# Autodesk Inventor assembly: Sink cabinet
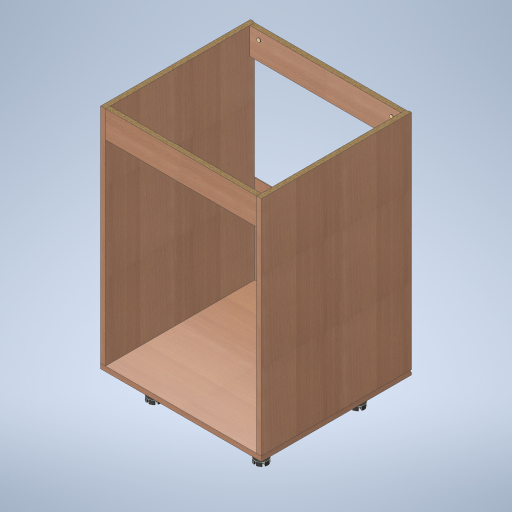
[picture p0: Inventor's stored thumbnail of the model, 512x512]
Saved by Autodesk Inventor 2024 (Build 280153000, 153)
## iProperties
RuleStatus: InUse
Created: 2017-01-27
Part Number: Sink cabinet
Document SubType Name: Assembly
Designer: SvetlanaB
Author: SvetlanaB
## Documents named in this file (17)
- C:\W4INV 2024 Design\iBOX LIBRARY\Kitchen\Standing Cabinets\Sink cabinet\Sink cabinet.iam
- C:\W4INV 2024 Design\iBOX LIBRARY\Kitchen\Standing Cabinets\Sink cabinet\Bottom panel.ipt
- C:\W4INV 2024 Design\iBOX LIBRARY\Kitchen\Standing Cabinets\Sink cabinet\Left panel.ipt
- C:\W4INV 2024 Design\iBOX LIBRARY\Kitchen\Standing Cabinets\Sink cabinet\Right panel.ipt
- C:\W4INV 2024 Design\iBOX LIBRARY\Kitchen\Standing Cabinets\Sink cabinet\Front panel.ipt
- C:\W4INV 2024 Design\iBOX LIBRARY\Kitchen\Standing Cabinets\Sink cabinet\Back top panel.ipt
- C:\W4INV 2024 Design\iBOX LIBRARY\Kitchen\Standing Cabinets\Sink cabinet\Back bottom panel.ipt
- C:\W4INV 2024 Design\_LIBRARY\Supports and legs\Legs\ADJUSTABLE LEG\Adjustable leg  BT18 clip included.ipt
- C:\W4INV 2024 Design\_LIBRARY\Supports and legs\Legs\ADJUSTABLE LEG\Adjustable leg  BT18.ipt
- C:\W4INV 2024 Design\_LIBRARY\Fixed joints\Confirmat\CONFIRMAT\Confirmat L50 NB T18 PB T 18.ipt
- C:\W4INV 2024 Design\iBOX LIBRARY\Kitchen\Standing Cabinets\Sink cabinet\Sink cabinet.ipt
- C:\W4INV 2024 Design\_LIBRARY\Fixed joints\Minifix joint\MINIFIX D15 v2\Minifix D15 & Dowel L34 & Cap D15 PB T18 LH.ipt
- C:\W4INV 2024 Design\_LIBRARY\Fixed joints\Minifix joint\MINIFIX D15 v2\Minifix D15 & Dowel L34 & Cap D15 PB T18 RH.ipt
- C:\W4INV 2024 Design\_LIBRARY\Fixed joints\Confirmat\CONFIRMAT\Confirmat L50 & Cap D10 NB T18 PB T 18.ipt
- C:\W4INV 2023 Design\LIBRARY\Fixed joints\Confirmat\CONFIRMAT.ipt
- C:\W4INV 2023 Design\LIBRARY\Fixed joints\Minifix joint\MINIFIX D15 v2.ipt
- C:\W4INV 2023 Design\LIBRARY\Supports and legs\Legs\ADJUSTABLE LEG.ipt
## Components (19 placed, 13 different names)
1. @Skeleton
2. Bottom panel:1 — Flush:1, Flush:2, Flush:3, Flush:4, Bottom board Plane:1, Front (Angle) Plane:1, Bottom board Plane:2, Front (Angle) Plane:2, Bottom board Plane:3, Front (Angle) Plane:3, Bottom board Plane:4, Front (Angle) Plane:4, Nestled Board Plane:1, Nestled Board Plane:2, Nestled Board Plane:3, Nestled Board Plane:4
3. Left panel:1 — Flush:5, Flush:6, Pillar Board Side Plane:2, Pillar Board Side Plane:4, Nestled Board Plane:5, Nestled Board Plane:8
4. Right panel:1 — Pillar Board Side Plane:1, Pillar Board Side Plane:3, Nestled Board Plane:6, Nestled Board Plane:7
5. Front panel:1 — Flush:11, Pillar Board Side Plane :1, Pillar Board Side Plane :2
6. Back top panel:1 — Pillar Board Side Plane :3, Pillar Board Side Plane :4
7. Back bottom panel:1
8. Adjustable leg  BT18 clip included:1 — Axis2 Plane:1, Bottom board Plane:1, Axis Plane:1, Front (Angle) Plane:1
9. Adjustable leg  BT18:2 — Axis2 Plane:2, Bottom board Plane:2, Axis Plane:2, Front (Angle) Plane:2
10. Adjustable leg  BT18 clip included:3 — Axis2 Plane:3, Bottom board Plane:3, Axis Plane:3, Front (Angle) Plane:3
11. Adjustable leg  BT18:4 — Axis2 Plane:4, Bottom board Plane:4, Axis Plane:4, Front (Angle) Plane:4
12. Confirmat L50 & Cap D10 NB T18 PB T 18:1 — Axis Plane:5, Pillar Board Side Plane:1, Nestled Board Plane:1
13. Confirmat L50 NB T18 PB T 18:2 — Axis Plane:6, Pillar Board Side Plane:2, Nestled Board Plane:2
14. Confirmat L50 NB T18 PB T 18:3 — Axis Plane:7, Pillar Board Side Plane:3, Nestled Board Plane:3
15. Confirmat L50 NB T18 PB T 18:4 — Axis Plane:8, Pillar Board Side Plane:4, Nestled Board Plane:4
16. Minifix D15 & Dowel L34 & Cap D15 PB T18 LH:1 — Nestled Board Plane:5, Pillar Board Side Plane :1, Axis Plane:9
17. Minifix D15 & Dowel L34 & Cap D15 PB T18 RH:2 — Nestled Board Plane:6, Pillar Board Side Plane :2, Axis Plane:10
18. Minifix D15 & Dowel L34 & Cap D15 PB T18 LH:3 — Axis Plane:11, Nestled Board Plane:7, Pillar Board Side Plane :3
19. Minifix D15 & Dowel L34 & Cap D15 PB T18 RH:4 — Nestled Board Plane:8, Pillar Board Side Plane :4, Axis Plane:12
## Relationships (47: Mate 28, Flush 15, Angle 4)
- Flush:1 (-100 mm): Bottom panel:1
- Flush:2 (-100 mm): Bottom panel:1
- Flush:3 (-100 mm): Bottom panel:1
- Flush:4 (-100 mm): Bottom panel:1
- Flush:5 (-64 mm): Left panel:1
- Flush:6 (-64 mm): Left panel:1
- Flush:11 (-30 mm): Front panel:1
- Axis2 Plane:1 [Mate]: Adjustable leg  BT18 clip included:1
- Bottom board Plane:1 [Mate]: Bottom panel:1 ↔ Adjustable leg  BT18 clip included:1
- Axis Plane:1 [Mate]: Adjustable leg  BT18 clip included:1
- Front (Angle) Plane:1 [Angle] (0 deg): Bottom panel:1 ↔ Adjustable leg  BT18 clip included:1
- Axis2 Plane:2 [Mate]: Adjustable leg  BT18:2
- Bottom board Plane:2 [Mate]: Bottom panel:1 ↔ Adjustable leg  BT18:2
- Axis Plane:2 [Mate]: Adjustable leg  BT18:2
- Front (Angle) Plane:2 [Angle] (0 deg): Bottom panel:1 ↔ Adjustable leg  BT18:2
- Axis2 Plane:3 [Mate]: Adjustable leg  BT18 clip included:3
- Bottom board Plane:3 [Mate]: Bottom panel:1 ↔ Adjustable leg  BT18 clip included:3
- Axis Plane:3 [Mate]: Adjustable leg  BT18 clip included:3
- Front (Angle) Plane:3 [Angle] (0 deg): Bottom panel:1 ↔ Adjustable leg  BT18 clip included:3
- Axis2 Plane:4 [Mate]: Adjustable leg  BT18:4
- Bottom board Plane:4 [Mate]: Bottom panel:1 ↔ Adjustable leg  BT18:4
- Axis Plane:4 [Mate]: Adjustable leg  BT18:4
- Front (Angle) Plane:4 [Angle] (0 deg): Bottom panel:1 ↔ Adjustable leg  BT18:4
- Axis Plane:5 [Mate]: Confirmat L50 & Cap D10 NB T18 PB T 18:1
- Pillar Board Side Plane:1 [Mate] (-9 mm): Right panel:1 ↔ Confirmat L50 & Cap D10 NB T18 PB T 18:1
- Nestled Board Plane:1 [Flush]: Bottom panel:1 ↔ Confirmat L50 & Cap D10 NB T18 PB T 18:1
- Axis Plane:6 [Mate]: Confirmat L50 NB T18 PB T 18:2
- Pillar Board Side Plane:2 [Mate] (-9 mm): Left panel:1 ↔ Confirmat L50 NB T18 PB T 18:2
- Nestled Board Plane:2 [Flush]: Bottom panel:1 ↔ Confirmat L50 NB T18 PB T 18:2
- Axis Plane:7 [Mate]: Confirmat L50 NB T18 PB T 18:3
- Pillar Board Side Plane:3 [Mate] (-9 mm): Right panel:1 ↔ Confirmat L50 NB T18 PB T 18:3
- Nestled Board Plane:3 [Flush]: Bottom panel:1 ↔ Confirmat L50 NB T18 PB T 18:3
- Axis Plane:8 [Mate]: Confirmat L50 NB T18 PB T 18:4
- Pillar Board Side Plane:4 [Mate] (-9 mm): Left panel:1 ↔ Confirmat L50 NB T18 PB T 18:4
- Nestled Board Plane:4 [Flush]: Bottom panel:1 ↔ Confirmat L50 NB T18 PB T 18:4
- Nestled Board Plane:5 [Mate]: Left panel:1 ↔ Minifix D15 & Dowel L34 & Cap D15 PB T18 LH:1
- Pillar Board Side Plane :1 [Flush] (18 mm): Front panel:1 ↔ Minifix D15 & Dowel L34 & Cap D15 PB T18 LH:1
- Axis Plane:9 [Mate]: Minifix D15 & Dowel L34 & Cap D15 PB T18 LH:1
- Nestled Board Plane:6 [Mate]: Right panel:1 ↔ Minifix D15 & Dowel L34 & Cap D15 PB T18 RH:2
- Pillar Board Side Plane :2 [Flush] (18 mm): Front panel:1 ↔ Minifix D15 & Dowel L34 & Cap D15 PB T18 RH:2
- Axis Plane:10 [Mate]: Minifix D15 & Dowel L34 & Cap D15 PB T18 RH:2
- Axis Plane:11 [Mate]: Minifix D15 & Dowel L34 & Cap D15 PB T18 LH:3
- Nestled Board Plane:7 [Mate]: Right panel:1 ↔ Minifix D15 & Dowel L34 & Cap D15 PB T18 LH:3
- Pillar Board Side Plane :3 [Flush] (18 mm): Back top panel:1 ↔ Minifix D15 & Dowel L34 & Cap D15 PB T18 LH:3
- Nestled Board Plane:8 [Mate]: Left panel:1 ↔ Minifix D15 & Dowel L34 & Cap D15 PB T18 RH:4
- Pillar Board Side Plane :4 [Flush] (18 mm): Back top panel:1 ↔ Minifix D15 & Dowel L34 & Cap D15 PB T18 RH:4
- Axis Plane:12 [Mate]: Minifix D15 & Dowel L34 & Cap D15 PB T18 RH:4
## Named parameters: Panel_thickness = 18 mm
